# Autodesk Inventor assembly: 1_Body
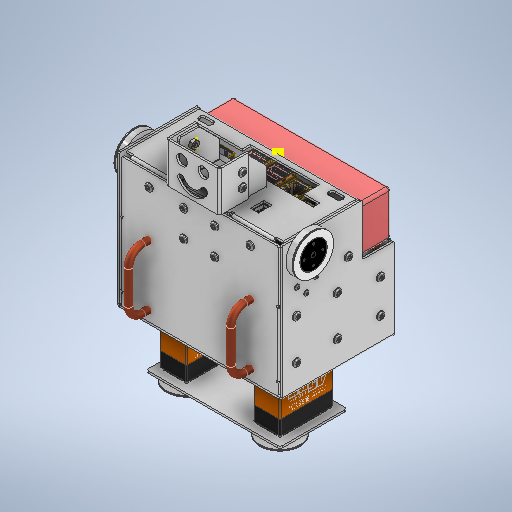
[picture p0: Inventor's stored thumbnail of the model, 512x512]
Saved by Autodesk Inventor 2026.1 (Build 301233000, 233)
## iProperties
Created: 2025-05-30
Part Number: 1_Body
Document SubType Name: Assembly
Designer: chris
Author: chris
## Documents named in this file (28)
- C:\Users\chris\Documents\Inventor\RHp_Humanoid_ver1\Assembly\1_Body.iam
- C:\Users\chris\Documents\Inventor\RHp_Humanoid_ver1\Part\Frame\Body\body_main_frame.ipt
- C:\Users\chris\Documents\Inventor\RHp_Humanoid_ver1\Part\Frame\Body\body_back_frame.ipt
- C:\Users\chris\Documents\Inventor\RHp_Humanoid_ver1\Part\Frame\Body\body_front_frame.ipt
- C:\Users\chris\Documents\Inventor\RHp_Humanoid_ver1\Part\Frame\Body\body_middle_frame.ipt
- C:\Users\chris\Documents\Inventor\RHp_Humanoid_ver1\Part\Frame\Body\body_motor_L_frame.ipt
- C:\Users\chris\Documents\Inventor\RHp_Humanoid_ver1\Part\Frame\Body\body_motor_R_frame.ipt
- C:\Users\chris\Documents\Inventor\RHp_Humanoid_ver1\Part\Frame\Body\body_top_frame.ipt
- C:\Users\chris\Documents\Inventor\RHp_Humanoid_ver1\Part\Other Parts\Servo_Driver.ipt
- C:\Users\chris\Documents\Inventor\RHp_Humanoid_ver1\Part\Other Parts\Battery_Pack.ipt
- C:\Users\chris\Documents\Inventor\RHp_Humanoid_ver1\Part\Other Parts\jetson_orin_super.ipt
- C:\Users\chris\Documents\Inventor\RHp_Humanoid_ver1\Part\HTD-45H, Horn\Horn\Top Horn.ipt
- C:\Users\chris\Documents\Inventor\RHp_Humanoid_ver1\Part\Frame\Body\body_bottom_frame.ipt
- C:\Users\chris\Documents\Inventor\RHp_Humanoid_ver1\Part\Other Parts\frame_motor_support_top_R.ipt
- C:\Users\chris\Documents\Inventor\RHp_Humanoid_ver1\Part\Other Parts\frame_motor_support_top_L.ipt
- C:\Users\chris\Documents\Inventor\RHp_Humanoid_ver1\Part\Bolt, Bearing, Nut, Washer\2030 Teflon Sheet.ipt
- C:\Users\chris\Documents\Inventor\RHp_Humanoid_ver1\Part\Other Parts\frame_support.ipt
- C:\Users\chris\Documents\Inventor\RHp_Humanoid_ver1\Part\HTD-45H, Horn\HTD-45H\HTD-45H.ipt
- C:\Users\chris\Documents\Inventor\RHp_Humanoid_ver1\Part\Other Parts\frame_motor_support_bottom_L.ipt
- C:\Users\chris\Documents\Inventor\RHp_Humanoid_ver1\Part\Other Parts\frame_motor_support_bottom_R.ipt
- C:\Users\chris\Documents\Inventor\RHp_Humanoid_ver1\Part\Bolt, Bearing, Nut, Washer\M3x6 Bolt.ipt
- C:\Users\chris\Documents\Inventor\RHp_Humanoid_ver1\Part\Bolt, Bearing, Nut, Washer\M3 Nut.ipt
- C:\Users\chris\Documents\Inventor\RHp_Humanoid_ver1\Part\Bolt, Bearing, Nut, Washer\M2x4 Bolt.ipt
- C:\Users\chris\Documents\Inventor\RHp_Humanoid_ver1\Part\Bolt, Bearing, Nut, Washer\M2x6 Bolt.ipt
- C:\Users\chris\Documents\Inventor\RHp_Humanoid_ver1\Part\Bolt, Bearing, Nut, Washer\M2x35 Bolt.ipt
- C:\Users\chris\Documents\Inventor\RHp_Humanoid_ver1\Part\HTD-45H, Horn\HTD-45H\M2x32.ipt
- C:\Users\chris\Documents\Inventor\RHp_Humanoid_ver1\Part\Frame\Head\Head1.ipt
- C:\Users\chris\Documents\Inventor\RHp_Humanoid_ver1\Part\Frame\Head\Head2.ipt
## Components (185 placed, 27 different names)
1. body_main_frame:1 — Mate:3, Flush:2, Mate:4, Mate:5, Flush:3, Flush:4, Mate:6, Flush:5, Mate:8, Mate:10, Mate:11, Flush:9, Flush:10, Mate:16, Mate:18, Flush:13, Mate:30, Flush:30, Flush:31, Mate:46, Mate:47, Mate:48, Mate:49, Mate:50, Mate:51, Mate:64, Mate:66, Mate:68, Flush:34, Flush:35, Mate:69, Flush:36, Flush:37, Rigid:25, Rigid:26, Rigid:29, Rigid:30, Rigid:33, Rigid:34, Rigid:35, Rigid:36, Rigid:41, Rigid:42, Rigid:65, Rigid:66, Rigid:67, Rigid:68, Rigid:73, Rigid:74, Rigid:75, Rigid:76, Rigid:77, Rigid:78, Rigid:99, Rigid:100, Rigid:101, Rigid:102, Rigid:103, Rigid:104, Rigid:105, Rigid:106, Rigid:107, Rigid:108, Rigid:109, Rigid:110
2. body_middle_frame:1 — Mate:6, Flush:5, Flush:6, Mate:17, Mate:28, Flush:29, Mate:29, Mate:65, Flush:32, Flush:33, Mate:67, Rigid:9, Rigid:10, Rigid:11, Rigid:12, Rigid:13, Rigid:14, Rigid:15, Rigid:16, Rigid:27, Rigid:28, Rigid:31, Rigid:32
3. body_front_frame:1 — Mate:5, Flush:3, Flush:4, Flush:6, Mate:7, Flush:7, Mate:9, Flush:8, Mate:58, Mate:59, Mate:60, Mate:61, Mate:62, Mate:63, Rigid:17, Rigid:18, Rigid:19, Rigid:20, Rigid:45, Rigid:46, Rigid:49, Rigid:50, Rigid:51, Rigid:52, Rigid:57, Rigid:58, Rigid:59, Rigid:60, Rigid:69, Rigid:70, Rigid:71, Rigid:72
4. body_back_frame:1 — Mate:3, Flush:2, Mate:4, Mate:19, Mate:52, Mate:53, Mate:54, Mate:55, Mate:56, Mate:57, Rigid:37, Rigid:38, Rigid:39, Rigid:40, Rigid:61, Rigid:62, Rigid:63, Rigid:64
5. body_top_frame:1 — Mate:11, Flush:9, Flush:10, Mate:20, Rigid:43, Rigid:44, Rigid:47, Rigid:48, Mate:89, Flush:91, Flush:92, Rigid:145, Rigid:146, Rigid:147, Rigid:148
6. body_bottom_frame:1 — Mate:80, Mate:81, Mate:82, Mate:83, Mate:84, Mate:85, Mate:86, Mate:87, Mate:88, Rigid:111, Rigid:112, Rigid:113, Rigid:114, Rigid:115, Rigid:116
7. Servo_Driver:1 — Mate:16, Mate:17, Mate:18, Rigid:1, Rigid:2, Rigid:3, Rigid:4
8. Battery_Pack:1 — Mate:19, Mate:20, Flush:13
9. jetson_orin_super:1 — Mate:28, Flush:29, Mate:29
10. M3x6 Bolt:41 — Rigid:133
11. M3x6 Bolt:42 — Rigid:134
12. M3x6 Bolt:43 — Rigid:140
13. M3x6 Bolt:44 — Rigid:139
14. M3x6 Bolt:45 — Rigid:136
15. M3x6 Bolt:46 — Rigid:135
16. M3x6 Bolt:47 — Rigid:138
17. M3x6 Bolt:48 — Rigid:137
18. M3 Nut:33 — Rigid:145
19. M3 Nut:34 — Rigid:146
20. M3 Nut:35 — Rigid:147
21. M3 Nut:36 — Rigid:148
22. M3 Nut:37 — Rigid:141
23. M3 Nut:38 — Rigid:142
24. M3 Nut:39 — Rigid:143
25. M3 Nut:40 — Rigid:144
26. Head1:1 — Mate:89, Flush:91, Flush:92, Mate:90, Mate:91, Mate:92, Rigid:135, Rigid:136, Rigid:137, Rigid:138, Rigid:141, Rigid:142, Rigid:143, Rigid:144
27. Head2:1 — Mate:90, Mate:91, Mate:92, Rigid:133, Rigid:134, Rigid:139, Rigid:140
28. HTD-45H:1 — Mate:69, Flush:36, Flush:37, Rotational:3, Mate:81, Rigid:127, Rigid:128
29. HTD-45H:2 — Mate:68, Flush:34, Flush:35, Rotational:4, Mate:80, Mate:82, Rigid:125, Rigid:126
30. HTD-45H:3 — Mate:66, Flush:33, Mate:67, Rotational:2, Rigid:129, Rigid:130
31. HTD-45H:4 — Mate:64, Mate:65, Flush:32, Rotational:1, Rigid:131, Rigid:132
32. Top Horn:1 — Rotational:2
33. Top Horn:2 — Rotational:1
34. 2030 Teflon Sheet:1 — Insert:1, Insert:2
35. 2030 Teflon Sheet:2 — Insert:2
36. 2030 Teflon Sheet:3 — Insert:3, Insert:4
37. 2030 Teflon Sheet:4 — Insert:4
38. frame_motor_support_top_R:1 — Mate:46, Mate:47, Mate:48, Insert:3, Rigid:81, Rigid:84, Rigid:85, Rigid:86
39. frame_motor_support_top_L:1 — Mate:49, Mate:50, Mate:51, Insert:1, Rigid:79, Rigid:80, Rigid:82, Rigid:83
40. body_motor_R_frame:1 — Mate:9, Mate:10, Flush:8, Rigid:5, Rigid:7, Rigid:22, Rigid:24, Rigid:53, Rigid:54, Rigid:87, Rigid:88, Rigid:89, Rigid:90, Rigid:91, Rigid:92
41. body_motor_L_frame:1 — Mate:7, Flush:7, Mate:8, Rigid:6, Rigid:8, Rigid:21, Rigid:23, Rigid:55, Rigid:56, Rigid:93, Rigid:94, Rigid:95, Rigid:96, Rigid:97, Rigid:98
42. M3x6 Bolt:9 — Rigid:17
43. M3x6 Bolt:10 — Rigid:20
44. M3x6 Bolt:11 — Rigid:18
45. M3x6 Bolt:12 — Rigid:19
46. M3x6 Bolt:13 — Rigid:29
47. M3x6 Bolt:14 — Rigid:30
48. M3x6 Bolt:15 — Rigid:26
49. M3x6 Bolt:16 — Rigid:25
50. M3 Nut:9 — Rigid:24
51. M3 Nut:10 — Rigid:23
52. M3 Nut:11 — Rigid:22
53. M3 Nut:12 — Rigid:21
54. M3 Nut:13 — Rigid:31
55. M3 Nut:14 — Rigid:32
56. M3 Nut:15 — Rigid:27
57. M3 Nut:16 — Rigid:28
58. M3x6 Bolt:1 — Rigid:4
59. M3x6 Bolt:2 — Rigid:3
60. M3x6 Bolt:3 — Rigid:2
61. M3x6 Bolt:4 — Rigid:1
62. M3x6 Bolt:5 — Rigid:5
63. M3x6 Bolt:6 — Rigid:6
64. M3x6 Bolt:7 — Rigid:7
65. M3x6 Bolt:8 — Rigid:8
66. M3 Nut:1 — Rigid:9
67. M3 Nut:2 — Rigid:10
68. M3 Nut:3 — Rigid:11
69. M3 Nut:4 — Rigid:12
70. M3 Nut:5 — Rigid:13
71. M3 Nut:6 — Rigid:14
72. M3 Nut:7 — Rigid:15
73. M3 Nut:8 — Rigid:16
74. frame_support:3 — Mate:59, Mate:61, Mate:63
75. frame_support:4 — Mate:58, Mate:60, Mate:62
76. M3x6 Bolt:37 — Rigid:66
77. M3x6 Bolt:38 — Rigid:65
78. M3x6 Bolt:39 — Rigid:68
79. M3x6 Bolt:40 — Rigid:67
80. M3 Nut:29 — Rigid:69
81. M3 Nut:30 — Rigid:70
82. M3 Nut:31 — Rigid:71
83. M3 Nut:32 — Rigid:72
84. M3x6 Bolt:29 — Rigid:57
85. M3x6 Bolt:30 — Rigid:58
86. M3x6 Bolt:31 — Rigid:60
87. M3x6 Bolt:32 — Rigid:59
88. M3x6 Bolt:25 — Rigid:49
89. M3x6 Bolt:26 — Rigid:51
90. M3x6 Bolt:27 — Rigid:50
91. M3x6 Bolt:28 — Rigid:52
92. M3 Nut:25 — Rigid:53
93. M3 Nut:26 — Rigid:55
94. M3 Nut:27 — Rigid:54
95. M3 Nut:28 — Rigid:56
96. frame_support:1 — Mate:52, Mate:53, Mate:54
97. frame_support:2 — Mate:55, Mate:56, Mate:57
98. M3x6 Bolt:33 — Rigid:61
99. M3x6 Bolt:34 — Rigid:62
100. M3x6 Bolt:35 — Rigid:64
101. M3x6 Bolt:36 — Rigid:63
102. M3x6 Bolt:17 — Rigid:33
103. M3x6 Bolt:18 — Rigid:35
104. M3x6 Bolt:19 — Rigid:34
105. M3x6 Bolt:20 — Rigid:36
106. M3 Nut:17 — Rigid:37
107. M3 Nut:18 — Rigid:38
108. M3 Nut:19 — Rigid:39
109. M3 Nut:20 — Rigid:40
110. M3x6 Bolt:21 — Rigid:41
111. M3x6 Bolt:22 — Rigid:42
112. M3 Nut:21 — Rigid:43
113. M3 Nut:22 — Rigid:44
114. M3x6 Bolt:23 — Rigid:45
115. M3x6 Bolt:24 — Rigid:46
116. M3 Nut:23 — Rigid:48
117. M3 Nut:24 — Rigid:47
118. frame_motor_support_bottom_R:1 — Mate:83, Mate:84, Mate:85, Insert:5, Rigid:119, Rigid:120, Rigid:121, Rigid:122
119. frame_motor_support_bottom_L:1 — Mate:86, Mate:87, Mate:88, Insert:7, Rigid:117, Rigid:118, Rigid:123, Rigid:124
120. 2030 Teflon Sheet:5 — Insert:8
121. 2030 Teflon Sheet:6 — Insert:7, Insert:8
122. 2030 Teflon Sheet:7 — Insert:6
123. 2030 Teflon Sheet:8 — Insert:5, Insert:6
124. Top Horn:3 — Rotational:3
125. Top Horn:4 — Rotational:4
126. M2x32:7 — Rigid:132
127. M2x32:8 — Rigid:131
128. M2x4 Bolt:7 — Rigid:87
129. M2x4 Bolt:8 — Rigid:89
130. M2x4 Bolt:9 — Rigid:91
131. M2x4 Bolt:10 — Rigid:88
132. M2x4 Bolt:11 — Rigid:90
133. M2x4 Bolt:12 — Rigid:92
134. M2x4 Bolt:4 — Rigid:77
135. M2x4 Bolt:5 — Rigid:78
136. M2x4 Bolt:6 — Rigid:76
137. M2x6 Bolt:3 — Rigid:81
138. M2x6 Bolt:4 — Rigid:86
139. M2x35 Bolt:3 — Rigid:84
140. M2x35 Bolt:4 — Rigid:85
141. M2x32:5 — Rigid:130
142. M2x32:6 — Rigid:129
143. M2x4 Bolt:13 — Rigid:93
144. M2x4 Bolt:14 — Rigid:98
145. M2x4 Bolt:15 — Rigid:97
146. M2x4 Bolt:16 — Rigid:94
147. M2x4 Bolt:17 — Rigid:95
148. M2x4 Bolt:18 — Rigid:96
149. M2x4 Bolt:1 — Rigid:73
150. M2x4 Bolt:2 — Rigid:74
151. M2x4 Bolt:3 — Rigid:75
152. M2x6 Bolt:1 — Rigid:79
153. M2x6 Bolt:2 — Rigid:80
154. M2x35 Bolt:1 — Rigid:82
155. M2x35 Bolt:2 — Rigid:83
156. M2x32:1 — Rigid:126
157. M2x32:2 — Rigid:125
158. M2x4 Bolt:34 — Rigid:114
159. M2x4 Bolt:35 — Rigid:116
160. M2x4 Bolt:36 — Rigid:115
161. M2x6 Bolt:7 — Rigid:119
162. M2x6 Bolt:8 — Rigid:120
163. M2x35 Bolt:5 — Rigid:121
164. M2x35 Bolt:6 — Rigid:122
165. M2x4 Bolt:19 — Rigid:99
166. M2x4 Bolt:20 — Rigid:100
167. M2x4 Bolt:21 — Rigid:101
168. M2x4 Bolt:22 — Rigid:104
169. M2x4 Bolt:23 — Rigid:103
170. M2x4 Bolt:24 — Rigid:102
171. M2x32:3 — Rigid:127
172. M2x32:4 — Rigid:128
173. M2x4 Bolt:31 — Rigid:111
174. M2x4 Bolt:32 — Rigid:112
175. M2x4 Bolt:33 — Rigid:113
176. M2x6 Bolt:5 — Rigid:117
177. M2x6 Bolt:6 — Rigid:118
178. M2x35 Bolt:7 — Rigid:123
179. M2x35 Bolt:8 — Rigid:124
180. M2x4 Bolt:25 — Rigid:110
181. M2x4 Bolt:26 — Rigid:109
182. M2x4 Bolt:27 — Rigid:108
183. M2x4 Bolt:28 — Rigid:107
184. M2x4 Bolt:29 — Rigid:106
185. M2x4 Bolt:30 — Rigid:105
## Relationships (235: WeldJoint 148, Mate 54, Flush 21, Insert 8, RevoluteJoint 4)
- Mate:3: body_main_frame:1 ↔ body_back_frame:1
- Flush:2: body_main_frame:1 ↔ body_back_frame:1
- Mate:4: body_main_frame:1 ↔ body_back_frame:1
- Mate:5: body_main_frame:1 ↔ body_front_frame:1
- Flush:3 (1.5 mm): body_main_frame:1 ↔ body_front_frame:1
- Flush:4: body_main_frame:1 ↔ body_front_frame:1
- Mate:6: body_main_frame:1 ↔ body_middle_frame:1
- Flush:5 (1.5 mm): body_main_frame:1 ↔ body_middle_frame:1
- Flush:6 (-30 mm): body_middle_frame:1 ↔ body_front_frame:1
- Mate:7: body_front_frame:1 ↔ body_motor_L_frame:1
- Flush:7: body_front_frame:1 ↔ body_motor_L_frame:1
- Mate:8 (40 mm): body_main_frame:1 ↔ body_motor_L_frame:1
- Mate:9: body_front_frame:1 ↔ body_motor_R_frame:1
- Mate:10 (40 mm): body_main_frame:1 ↔ body_motor_R_frame:1
- Mate:11: body_main_frame:1 ↔ body_top_frame:1
- Flush:8: body_front_frame:1 ↔ body_motor_R_frame:1
- Flush:9: body_main_frame:1 ↔ body_top_frame:1
- Flush:10 (1.5 mm): body_main_frame:1 ↔ body_top_frame:1
- Mate:16 (10 mm): body_main_frame:1 ↔ Servo_Driver:1
- Mate:17: body_middle_frame:1 ↔ Servo_Driver:1
- Mate:18 (31 mm): body_main_frame:1 ↔ Servo_Driver:1
- Mate:19: body_back_frame:1 ↔ Battery_Pack:1
- Mate:20: body_top_frame:1 ↔ Battery_Pack:1
- Flush:13 (-2.5 mm): body_main_frame:1 ↔ Battery_Pack:1
- Mate:28: body_middle_frame:1 ↔ jetson_orin_super:1
- Flush:29 (6 mm): body_middle_frame:1 ↔ jetson_orin_super:1
- Mate:29 (7 mm): body_middle_frame:1 ↔ jetson_orin_super:1
- Mate:30: body_main_frame:1
- Flush:30: body_main_frame:1
- Flush:31: body_main_frame:1
- Mate:46: body_main_frame:1 ↔ frame_motor_support_top_R:1
- Mate:47: body_main_frame:1 ↔ frame_motor_support_top_R:1
- Mate:48: body_main_frame:1 ↔ frame_motor_support_top_R:1
- Mate:49: body_main_frame:1 ↔ frame_motor_support_top_L:1
- Mate:50: body_main_frame:1 ↔ frame_motor_support_top_L:1
- Mate:51: body_main_frame:1 ↔ frame_motor_support_top_L:1
- Insert:1: 2030 Teflon Sheet:1 ↔ frame_motor_support_top_L:1
- Insert:2 (0.07 mm): 2030 Teflon Sheet:1 ↔ 2030 Teflon Sheet:2
- Insert:3: 2030 Teflon Sheet:3 ↔ frame_motor_support_top_R:1
- Insert:4 (0.07 mm): 2030 Teflon Sheet:3 ↔ 2030 Teflon Sheet:4
- Mate:52: body_back_frame:1 ↔ frame_support:1
- Mate:53: body_back_frame:1 ↔ frame_support:1
- Mate:54: body_back_frame:1 ↔ frame_support:1
- Mate:55: body_back_frame:1 ↔ frame_support:2
- Mate:56: body_back_frame:1 ↔ frame_support:2
- Mate:57: body_back_frame:1 ↔ frame_support:2
- Mate:58: body_front_frame:1 ↔ frame_support:4
- Mate:59: body_front_frame:1 ↔ frame_support:3
- Mate:60: body_front_frame:1 ↔ frame_support:4
- Mate:61: body_front_frame:1 ↔ frame_support:3
- Mate:62: body_front_frame:1 ↔ frame_support:4
- Mate:63: body_front_frame:1 ↔ frame_support:3
- Mate:64: body_main_frame:1 ↔ HTD-45H:4
- Mate:65 (2 mm): body_middle_frame:1 ↔ HTD-45H:4
- Flush:32: body_middle_frame:1 ↔ HTD-45H:4
- Mate:66: body_main_frame:1 ↔ HTD-45H:3
- Flush:33: body_middle_frame:1 ↔ HTD-45H:3
- Mate:67 (2 mm): body_middle_frame:1 ↔ HTD-45H:3
- Mate:68: body_main_frame:1 ↔ HTD-45H:2
- Flush:34 (15 mm): body_main_frame:1 ↔ HTD-45H:2
- Flush:35 (16.5 mm): body_main_frame:1 ↔ HTD-45H:2
- Mate:69: body_main_frame:1 ↔ HTD-45H:1
- Flush:36 (15 mm): body_main_frame:1 ↔ HTD-45H:1
- Flush:37 (16.5 mm): body_main_frame:1 ↔ HTD-45H:1
- Rotational:1 [RevoluteJoint]: HTD-45H:4 ↔ Top Horn:2
- Rotational:2 [RevoluteJoint]: HTD-45H:3 ↔ Top Horn:1
- Rotational:3 [RevoluteJoint]: HTD-45H:1 ↔ Top Horn:3
- Rotational:4 [RevoluteJoint]: HTD-45H:2 ↔ Top Horn:4
- Mate:80: body_bottom_frame:1 ↔ HTD-45H:2
- Mate:81: body_bottom_frame:1 ↔ HTD-45H:1
- Mate:82: body_bottom_frame:1 ↔ HTD-45H:2
- Mate:83: body_bottom_frame:1 ↔ frame_motor_support_bottom_R:1
- Mate:84: body_bottom_frame:1 ↔ frame_motor_support_bottom_R:1
- Mate:85: body_bottom_frame:1 ↔ frame_motor_support_bottom_R:1
- Mate:86: body_bottom_frame:1 ↔ frame_motor_support_bottom_L:1
- Mate:87: body_bottom_frame:1 ↔ frame_motor_support_bottom_L:1
- Mate:88: body_bottom_frame:1 ↔ frame_motor_support_bottom_L:1
- Insert:5: frame_motor_support_bottom_R:1 ↔ 2030 Teflon Sheet:8
- Insert:6 (0.07 mm): 2030 Teflon Sheet:7 ↔ 2030 Teflon Sheet:8
- Insert:7: frame_motor_support_bottom_L:1 ↔ 2030 Teflon Sheet:6
- Insert:8 (0.07 mm): 2030 Teflon Sheet:5 ↔ 2030 Teflon Sheet:6
- Rigid:1 [WeldJoint]: Servo_Driver:1 ↔ M3x6 Bolt:4
- Rigid:2 [WeldJoint]: Servo_Driver:1 ↔ M3x6 Bolt:3
- Rigid:3 [WeldJoint]: Servo_Driver:1 ↔ M3x6 Bolt:2
- Rigid:4 [WeldJoint]: Servo_Driver:1 ↔ M3x6 Bolt:1
- Rigid:5 [WeldJoint]: body_motor_R_frame:1 ↔ M3x6 Bolt:5
- Rigid:6 [WeldJoint]: body_motor_L_frame:1 ↔ M3x6 Bolt:6
- Rigid:7 [WeldJoint]: body_motor_R_frame:1 ↔ M3x6 Bolt:7
- Rigid:8 [WeldJoint]: body_motor_L_frame:1 ↔ M3x6 Bolt:8
- Rigid:9 [WeldJoint]: body_middle_frame:1 ↔ M3 Nut:1
- Rigid:10 [WeldJoint]: body_middle_frame:1 ↔ M3 Nut:2
- Rigid:11 [WeldJoint]: body_middle_frame:1 ↔ M3 Nut:3
- Rigid:12 [WeldJoint]: body_middle_frame:1 ↔ M3 Nut:4
- Rigid:13 [WeldJoint]: body_middle_frame:1 ↔ M3 Nut:5
- Rigid:14 [WeldJoint]: body_middle_frame:1 ↔ M3 Nut:6
- Rigid:15 [WeldJoint]: body_middle_frame:1 ↔ M3 Nut:7
- Rigid:16 [WeldJoint]: body_middle_frame:1 ↔ M3 Nut:8
- Rigid:17 [WeldJoint]: body_front_frame:1 ↔ M3x6 Bolt:9
- Rigid:18 [WeldJoint]: body_front_frame:1 ↔ M3x6 Bolt:11
- Rigid:19 [WeldJoint]: body_front_frame:1 ↔ M3x6 Bolt:12
- Rigid:20 [WeldJoint]: body_front_frame:1 ↔ M3x6 Bolt:10
- Rigid:21 [WeldJoint]: body_motor_L_frame:1 ↔ M3 Nut:12
- Rigid:22 [WeldJoint]: body_motor_R_frame:1 ↔ M3 Nut:11
- Rigid:23 [WeldJoint]: body_motor_L_frame:1 ↔ M3 Nut:10
- Rigid:24 [WeldJoint]: body_motor_R_frame:1 ↔ M3 Nut:9
- Rigid:25 [WeldJoint]: body_main_frame:1 ↔ M3x6 Bolt:16
- Rigid:26 [WeldJoint]: body_main_frame:1 ↔ M3x6 Bolt:15
- Rigid:27 [WeldJoint]: body_middle_frame:1 ↔ M3 Nut:15
- Rigid:28 [WeldJoint]: body_middle_frame:1 ↔ M3 Nut:16
- Rigid:29 [WeldJoint]: body_main_frame:1 ↔ M3x6 Bolt:13
- Rigid:30 [WeldJoint]: body_main_frame:1 ↔ M3x6 Bolt:14
- Rigid:31 [WeldJoint]: body_middle_frame:1 ↔ M3 Nut:13
- Rigid:32 [WeldJoint]: body_middle_frame:1 ↔ M3 Nut:14
- Rigid:33 [WeldJoint]: body_main_frame:1 ↔ M3x6 Bolt:17
- Rigid:34 [WeldJoint]: body_main_frame:1 ↔ M3x6 Bolt:19
- Rigid:35 [WeldJoint]: body_main_frame:1 ↔ M3x6 Bolt:18
- Rigid:36 [WeldJoint]: body_main_frame:1 ↔ M3x6 Bolt:20
- Rigid:37 [WeldJoint]: body_back_frame:1 ↔ M3 Nut:17
- Rigid:38 [WeldJoint]: body_back_frame:1 ↔ M3 Nut:18
- Rigid:39 [WeldJoint]: body_back_frame:1 ↔ M3 Nut:19
- Rigid:40 [WeldJoint]: body_back_frame:1 ↔ M3 Nut:20
- Rigid:41 [WeldJoint]: body_main_frame:1 ↔ M3x6 Bolt:21
- Rigid:42 [WeldJoint]: body_main_frame:1 ↔ M3x6 Bolt:22
- Rigid:43 [WeldJoint]: body_top_frame:1 ↔ M3 Nut:21
- Rigid:44 [WeldJoint]: body_top_frame:1 ↔ M3 Nut:22
- Rigid:45 [WeldJoint]: body_front_frame:1 ↔ M3x6 Bolt:23
- Rigid:46 [WeldJoint]: body_front_frame:1 ↔ M3x6 Bolt:24
- Rigid:47 [WeldJoint]: body_top_frame:1 ↔ M3 Nut:24
- Rigid:48 [WeldJoint]: body_top_frame:1 ↔ M3 Nut:23
- Rigid:49 [WeldJoint]: body_front_frame:1 ↔ M3x6 Bolt:25
- Rigid:50 [WeldJoint]: body_front_frame:1 ↔ M3x6 Bolt:27
- Rigid:51 [WeldJoint]: body_front_frame:1 ↔ M3x6 Bolt:26
- Rigid:52 [WeldJoint]: body_front_frame:1 ↔ M3x6 Bolt:28
- Rigid:53 [WeldJoint]: body_motor_R_frame:1 ↔ M3 Nut:25
- Rigid:54 [WeldJoint]: body_motor_R_frame:1 ↔ M3 Nut:27
- Rigid:55 [WeldJoint]: body_motor_L_frame:1 ↔ M3 Nut:26
- Rigid:56 [WeldJoint]: body_motor_L_frame:1 ↔ M3 Nut:28
- Rigid:57 [WeldJoint]: body_front_frame:1 ↔ M3x6 Bolt:29
- Rigid:58 [WeldJoint]: body_front_frame:1 ↔ M3x6 Bolt:30
- Rigid:59 [WeldJoint]: body_front_frame:1 ↔ M3x6 Bolt:32
- Rigid:60 [WeldJoint]: body_front_frame:1 ↔ M3x6 Bolt:31
- Rigid:61 [WeldJoint]: body_back_frame:1 ↔ M3x6 Bolt:33
- Rigid:62 [WeldJoint]: body_back_frame:1 ↔ M3x6 Bolt:34
- Rigid:63 [WeldJoint]: body_back_frame:1 ↔ M3x6 Bolt:36
- Rigid:64 [WeldJoint]: body_back_frame:1 ↔ M3x6 Bolt:35
- Rigid:65 [WeldJoint]: body_main_frame:1 ↔ M3x6 Bolt:38
- Rigid:66 [WeldJoint]: body_main_frame:1 ↔ M3x6 Bolt:37
- Rigid:67 [WeldJoint]: body_main_frame:1 ↔ M3x6 Bolt:40
- Rigid:68 [WeldJoint]: body_main_frame:1 ↔ M3x6 Bolt:39
- Rigid:69 [WeldJoint]: body_front_frame:1 ↔ M3 Nut:29
- Rigid:70 [WeldJoint]: body_front_frame:1 ↔ M3 Nut:30
- Rigid:71 [WeldJoint]: body_front_frame:1 ↔ M3 Nut:31
- Rigid:72 [WeldJoint]: body_front_frame:1 ↔ M3 Nut:32
- Rigid:73 [WeldJoint]: body_main_frame:1 ↔ M2x4 Bolt:1
- Rigid:74 [WeldJoint]: body_main_frame:1 ↔ M2x4 Bolt:2
- Rigid:75 [WeldJoint]: body_main_frame:1 ↔ M2x4 Bolt:3
- Rigid:76 [WeldJoint]: body_main_frame:1 ↔ M2x4 Bolt:6
- Rigid:77 [WeldJoint]: body_main_frame:1 ↔ M2x4 Bolt:4
- Rigid:78 [WeldJoint]: body_main_frame:1 ↔ M2x4 Bolt:5
- Rigid:79 [WeldJoint]: frame_motor_support_top_L:1 ↔ M2x6 Bolt:1
- Rigid:80 [WeldJoint]: frame_motor_support_top_L:1 ↔ M2x6 Bolt:2
- Rigid:81 [WeldJoint]: frame_motor_support_top_R:1 ↔ M2x6 Bolt:3
- Rigid:82 [WeldJoint]: frame_motor_support_top_L:1 ↔ M2x35 Bolt:1
- Rigid:83 [WeldJoint]: frame_motor_support_top_L:1 ↔ M2x35 Bolt:2
- Rigid:84 [WeldJoint]: frame_motor_support_top_R:1 ↔ M2x35 Bolt:3
- Rigid:85 [WeldJoint]: frame_motor_support_top_R:1 ↔ M2x35 Bolt:4
- Rigid:86 [WeldJoint]: frame_motor_support_top_R:1 ↔ M2x6 Bolt:4
- Rigid:87 [WeldJoint]: body_motor_R_frame:1 ↔ M2x4 Bolt:7
- Rigid:88 [WeldJoint]: body_motor_R_frame:1 ↔ M2x4 Bolt:10
- Rigid:89 [WeldJoint]: body_motor_R_frame:1 ↔ M2x4 Bolt:8
- Rigid:90 [WeldJoint]: body_motor_R_frame:1 ↔ M2x4 Bolt:11
- Rigid:91 [WeldJoint]: body_motor_R_frame:1 ↔ M2x4 Bolt:9
- Rigid:92 [WeldJoint]: body_motor_R_frame:1 ↔ M2x4 Bolt:12
- Rigid:93 [WeldJoint]: body_motor_L_frame:1 ↔ M2x4 Bolt:13
- Rigid:94 [WeldJoint]: body_motor_L_frame:1 ↔ M2x4 Bolt:16
- Rigid:95 [WeldJoint]: body_motor_L_frame:1 ↔ M2x4 Bolt:17
- Rigid:96 [WeldJoint]: body_motor_L_frame:1 ↔ M2x4 Bolt:18
- Rigid:97 [WeldJoint]: body_motor_L_frame:1 ↔ M2x4 Bolt:15
- Rigid:98 [WeldJoint]: body_motor_L_frame:1 ↔ M2x4 Bolt:14
- Rigid:99 [WeldJoint]: body_main_frame:1 ↔ M2x4 Bolt:19
- Rigid:100 [WeldJoint]: body_main_frame:1 ↔ M2x4 Bolt:20
- Rigid:101 [WeldJoint]: body_main_frame:1 ↔ M2x4 Bolt:21
- Rigid:102 [WeldJoint]: body_main_frame:1 ↔ M2x4 Bolt:24
- Rigid:103 [WeldJoint]: body_main_frame:1 ↔ M2x4 Bolt:23
- Rigid:104 [WeldJoint]: body_main_frame:1 ↔ M2x4 Bolt:22
- Rigid:105 [WeldJoint]: body_main_frame:1 ↔ M2x4 Bolt:30
- Rigid:106 [WeldJoint]: body_main_frame:1 ↔ M2x4 Bolt:29
- Rigid:107 [WeldJoint]: body_main_frame:1 ↔ M2x4 Bolt:28
- Rigid:108 [WeldJoint]: body_main_frame:1 ↔ M2x4 Bolt:27
- Rigid:109 [WeldJoint]: body_main_frame:1 ↔ M2x4 Bolt:26
- Rigid:110 [WeldJoint]: body_main_frame:1 ↔ M2x4 Bolt:25
- Rigid:111 [WeldJoint]: body_bottom_frame:1 ↔ M2x4 Bolt:31
- Rigid:112 [WeldJoint]: body_bottom_frame:1 ↔ M2x4 Bolt:32
- Rigid:113 [WeldJoint]: body_bottom_frame:1 ↔ M2x4 Bolt:33
- Rigid:114 [WeldJoint]: body_bottom_frame:1 ↔ M2x4 Bolt:34
- Rigid:115 [WeldJoint]: body_bottom_frame:1 ↔ M2x4 Bolt:36
- Rigid:116 [WeldJoint]: body_bottom_frame:1 ↔ M2x4 Bolt:35
- Rigid:117 [WeldJoint]: frame_motor_support_bottom_L:1 ↔ M2x6 Bolt:5
- Rigid:118 [WeldJoint]: frame_motor_support_bottom_L:1 ↔ M2x6 Bolt:6
- Rigid:119 [WeldJoint]: frame_motor_support_bottom_R:1 ↔ M2x6 Bolt:7
- Rigid:120 [WeldJoint]: frame_motor_support_bottom_R:1 ↔ M2x6 Bolt:8
- Rigid:121 [WeldJoint]: frame_motor_support_bottom_R:1 ↔ M2x35 Bolt:5
- Rigid:122 [WeldJoint]: frame_motor_support_bottom_R:1 ↔ M2x35 Bolt:6
- Rigid:123 [WeldJoint]: frame_motor_support_bottom_L:1 ↔ M2x35 Bolt:7
- Rigid:124 [WeldJoint]: frame_motor_support_bottom_L:1 ↔ M2x35 Bolt:8
- Rigid:125 [WeldJoint]: HTD-45H:2 ↔ M2x32:2
- Rigid:126 [WeldJoint]: HTD-45H:2 ↔ M2x32:1
- Rigid:127 [WeldJoint]: HTD-45H:1 ↔ M2x32:3
- Rigid:128 [WeldJoint]: HTD-45H:1 ↔ M2x32:4
- Rigid:129 [WeldJoint]: HTD-45H:3 ↔ M2x32:6
- Rigid:130 [WeldJoint]: HTD-45H:3 ↔ M2x32:5
- Rigid:131 [WeldJoint]: HTD-45H:4 ↔ M2x32:8
- Rigid:132 [WeldJoint]: HTD-45H:4 ↔ M2x32:7
- Mate:89: body_top_frame:1 ↔ Head1:1
- Flush:91: body_top_frame:1 ↔ Head1:1
- Flush:92 (40 mm): body_top_frame:1 ↔ Head1:1
- Mate:90: Head1:1 ↔ Head2:1
- Mate:91 (0.31 mm): Head1:1 ↔ Head2:1
- Mate:92: Head1:1 ↔ Head2:1
- Rigid:133 [WeldJoint]: M3x6 Bolt:41 ↔ Head2:1
- Rigid:134 [WeldJoint]: M3x6 Bolt:42 ↔ Head2:1
- Rigid:135 [WeldJoint]: M3x6 Bolt:46 ↔ Head1:1
- Rigid:136 [WeldJoint]: M3x6 Bolt:45 ↔ Head1:1
- Rigid:137 [WeldJoint]: M3x6 Bolt:48 ↔ Head1:1
- Rigid:138 [WeldJoint]: M3x6 Bolt:47 ↔ Head1:1
- Rigid:139 [WeldJoint]: M3x6 Bolt:44 ↔ Head2:1
- Rigid:140 [WeldJoint]: M3x6 Bolt:43 ↔ Head2:1
- Rigid:141 [WeldJoint]: M3 Nut:37 ↔ Head1:1
- Rigid:142 [WeldJoint]: M3 Nut:38 ↔ Head1:1
- Rigid:143 [WeldJoint]: M3 Nut:39 ↔ Head1:1
- Rigid:144 [WeldJoint]: M3 Nut:40 ↔ Head1:1
- Rigid:145 [WeldJoint]: body_top_frame:1 ↔ M3 Nut:33
- Rigid:146 [WeldJoint]: body_top_frame:1 ↔ M3 Nut:34
- Rigid:147 [WeldJoint]: body_top_frame:1 ↔ M3 Nut:35
- Rigid:148 [WeldJoint]: body_top_frame:1 ↔ M3 Nut:36
